# Autodesk Inventor assembly: Assembly1
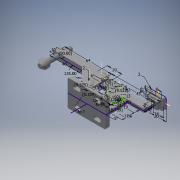
[picture p0: Inventor's stored thumbnail of the model, 180x180]
Saved by Autodesk Inventor 2018 (Build 220112000, 112)
## iProperties
Created: 2018-12-03
Part Number: Assembly1
Document SubType Name: Assembly
Designer: Jerry
Author: Jerry
## Documents named in this file (9)
- C:\Users\Jerry\OneDrive\Desktop\e25 sketchy inventor\last homework\Assembly1.iam
- C:\Users\Jerry\OneDrive\Desktop\e25 sketchy inventor\last homework\newfrontpart.ipt
- C:\Users\Jerry\OneDrive\Desktop\e25 sketchy inventor\last homework\rivet.ipt
- C:\Users\Jerry\OneDrive\Desktop\e25 sketchy inventor\last homework\tappy.ipt
- C:\Users\Jerry\OneDrive\Desktop\e25 sketchy inventor\last homework\basepart.ipt
- C:\Users\Jerry\OneDrive\Desktop\e25 sketchy inventor\last homework\smallthing.ipt
- C:\Users\Jerry\OneDrive\Desktop\e25 sketchy inventor\last homework\dick.ipt
- C:\Users\Jerry\OneDrive\Desktop\e25 sketchy inventor\last homework\dickhead.ipt
- C:\Users\Jerry\OneDrive\Desktop\e25 sketchy inventor\last homework\slab.ipt
## Components (12 placed, 8 different names)
1. newfrontpart:1 — Cylindrical:1, Cylindrical:2, Mate:1, Mate:2, Mate:5, Mate:6, Cylindrical:11
2. rivet:1 — Cylindrical:1, Cylindrical:3, Mate:5
3. rivet:2 — Cylindrical:6, Cylindrical:8, Cylindrical:10, Mate:8
4. rivet:3 — Cylindrical:2, Cylindrical:5, Mate:6
5. rivet:4 — Cylindrical:4, Cylindrical:7, Cylindrical:9, Mate:7
6. tappy:1 — Cylindrical:3, Mate:1, Cylindrical:4, Mate:3, Mate:4, Mate:10, Mate:11, Mate:12
7. basepart:1 — Cylindrical:5, Mate:2, Cylindrical:6
8. smallthing:1 — Cylindrical:7, Cylindrical:8, Mate:3, Mate:7, Mate:8
9. smallthing:2 — Cylindrical:9, Cylindrical:10, Mate:4
10. dick:1 — Cylindrical:11, Cylindrical:12, Mate:9
11. dickhead:1 — Cylindrical:12, Mate:9
12. slab:1 — Mate:10, Mate:11, Mate:12
## Relationships (24: CylindricalJoint 12, Mate 12)
- Cylindrical:1: newfrontpart:1 ↔ rivet:1
- Cylindrical:2: newfrontpart:1 ↔ rivet:3
- Cylindrical:3: rivet:1 ↔ tappy:1
- Mate:1: newfrontpart:1 ↔ tappy:1
- Cylindrical:4: rivet:4 ↔ tappy:1
- Cylindrical:5: rivet:3 ↔ basepart:1
- Mate:2: newfrontpart:1 ↔ basepart:1
- Cylindrical:6: rivet:2 ↔ basepart:1
- Cylindrical:7: rivet:4 ↔ smallthing:1
- Cylindrical:8: rivet:2 ↔ smallthing:1
- Cylindrical:9: rivet:4 ↔ smallthing:2
- Cylindrical:10: rivet:2 ↔ smallthing:2
- Mate:3: tappy:1 ↔ smallthing:1
- Mate:4: tappy:1 ↔ smallthing:2
- Mate:5: newfrontpart:1 ↔ rivet:1
- Mate:6: newfrontpart:1 ↔ rivet:3
- Mate:7: rivet:4 ↔ smallthing:1
- Mate:8: rivet:2 ↔ smallthing:1
- Cylindrical:11: newfrontpart:1 ↔ dick:1
- Cylindrical:12: dick:1 ↔ dickhead:1
- Mate:9: dick:1 ↔ dickhead:1
- Mate:10: tappy:1 ↔ slab:1
- Mate:11: tappy:1 ↔ slab:1
- Mate:12: tappy:1 ↔ slab:1
